# Autodesk Inventor assembly: Milestione One Assembly
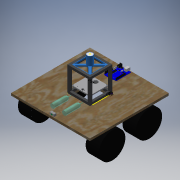
[picture p0: Inventor's stored thumbnail of the model, 180x180]
Saved by Autodesk Inventor 2016 (Build 200138000, 138)
## iProperties
Created: 2016-02-22
Part Number: Milestione One Assembly
Document SubType Name: Assembly
Designer: Kenneth Daniel
Author: Kenneth Daniel
## Documents named in this file (12)
- C:\Users\Kenneth Daniel\Documents\Enes 100A\CAD Assignments\Milestione One Assembly.iam
- C:\Users\Kenneth Daniel\Documents\Enes 100A\Bassic Vehicle Chassis.ipt
- C:\Users\Kenneth Daniel\Documents\Enes 100A\Lifting Main Frame.ipt
- C:\Users\Kenneth Daniel\Documents\Enes 100A\Motor housing for Lifting Platform.ipt
- C:\Users\Kenneth Daniel\Documents\Enes 100A\Moving Surface.ipt
- C:\Users\Kenneth Daniel\Documents\Enes 100A\Syringe Ken.ipt
- C:\Users\Kenneth Daniel\Documents\Enes 100A\CAD Assignments\Lifting Pad Motor Redo.ipt
- C:\Users\Kenneth Daniel\Documents\Enes 100A\CAD Assignments\Wheel Holder.ipt
- C:\Users\Kenneth Daniel\Documents\Enes 100A\CAD Assignments\Susspension Holder.ipt
- C:\Users\Kenneth Daniel\Documents\Enes 100A\CAD Assignments\Basic OSV Wheel.ipt
- C:\Users\Kenneth Daniel\Documents\Enes 100A\arduino uno.iam
- C:\Users\Kenneth Daniel\Documents\Enes 100A\CAD Assignments\Basic Sensor.ipt
## Components (25 placed, 11 different names)
1. Bassic Vehicle Chassis:1 — Mate:3, Mate:4, Mate:5, Mate:10, Mate:11, Mate:12, Mate:13, Mate:14, Mate:15, Mate:16, Mate:17, Mate:18, Mate:19, Mate:20, Mate:21, Mate:22, Mate:23, Mate:24, Mate:25, Mate:26, Mate:47
2. Lifting Main Frame:1 — Mate:1, Mate:2, Mate:3, Mate:4, Mate:5, Mate:6, Mate:7, Mate:8
3. Motor housing for Lifting Platform:1 — Mate:1, Mate:2, Mate:6, Mate:9
4. Moving Surface:1 — Mate:7, Mate:8
5. Syringe Ken:1
6. Syringe Ken:2
7. Lifting Pad Motor Redo:1 — Mate:9
8. Wheel Holder:1 — Mate:13, Mate:29, Mate:32, Mate:34, Mate:41, Mate:42
9. Wheel Holder:2 — Mate:12, Mate:28, Mate:37, Mate:38, Mate:45, Mate:46
10. Wheel Holder:3 — Mate:11, Mate:26, Mate:27, Mate:35, Mate:36, Mate:43, Mate:44
11. Wheel Holder:4 — Mate:10, Mate:30, Mate:31, Mate:33, Mate:39, Mate:40
12. Susspension Holder:1 — Mate:14, Mate:15, Mate:16, Mate:30
13. Susspension Holder:2 — Mate:17, Mate:18, Mate:19, Mate:29
14. Susspension Holder:3 — Mate:20, Mate:21, Mate:22, Mate:27
15. Susspension Holder:4 — Mate:23, Mate:24, Mate:25, Mate:28
16. Basic OSV Wheel:1 — Mate:31, Mate:33
17. Basic OSV Wheel:2 — Mate:35, Mate:36
18. Basic OSV Wheel:3 — Mate:32, Mate:34
19. Basic OSV Wheel:4 — Mate:37, Mate:38
20. Lifting Pad Motor Redo:2 — Mate:41, Mate:42
21. Lifting Pad Motor Redo:3 — Mate:39, Mate:40
22. Lifting Pad Motor Redo:4 — Mate:43, Mate:44
23. Lifting Pad Motor Redo:5 — Mate:45, Mate:46
24. arduino uno:1 [sub-assembly]
25. Basic Sensor:1 — Mate:47
## Relationships (47: Mate 47)
- Mate:1: Lifting Main Frame:1 ↔ Motor housing for Lifting Platform:1
- Mate:2: Lifting Main Frame:1 ↔ Motor housing for Lifting Platform:1
- Mate:3: Bassic Vehicle Chassis:1 ↔ Lifting Main Frame:1
- Mate:4: Bassic Vehicle Chassis:1 ↔ Lifting Main Frame:1
- Mate:5: Bassic Vehicle Chassis:1 ↔ Lifting Main Frame:1
- Mate:6: Lifting Main Frame:1 ↔ Motor housing for Lifting Platform:1
- Mate:7: Lifting Main Frame:1 ↔ Moving Surface:1
- Mate:8: Lifting Main Frame:1 ↔ Moving Surface:1
- Mate:9: Motor housing for Lifting Platform:1 ↔ Lifting Pad Motor Redo:1
- Mate:10: Bassic Vehicle Chassis:1 ↔ Wheel Holder:4
- Mate:11: Bassic Vehicle Chassis:1 ↔ Wheel Holder:3
- Mate:12: Bassic Vehicle Chassis:1 ↔ Wheel Holder:2
- Mate:13: Bassic Vehicle Chassis:1 ↔ Wheel Holder:1
- Mate:14: Bassic Vehicle Chassis:1 ↔ Susspension Holder:1
- Mate:15: Bassic Vehicle Chassis:1 ↔ Susspension Holder:1
- Mate:16: Bassic Vehicle Chassis:1 ↔ Susspension Holder:1
- Mate:17: Bassic Vehicle Chassis:1 ↔ Susspension Holder:2
- Mate:18: Bassic Vehicle Chassis:1 ↔ Susspension Holder:2
- Mate:19: Bassic Vehicle Chassis:1 ↔ Susspension Holder:2
- Mate:20: Bassic Vehicle Chassis:1 ↔ Susspension Holder:3
- Mate:21: Bassic Vehicle Chassis:1 ↔ Susspension Holder:3
- Mate:22: Bassic Vehicle Chassis:1 ↔ Susspension Holder:3
- Mate:23: Bassic Vehicle Chassis:1 ↔ Susspension Holder:4
- Mate:24: Bassic Vehicle Chassis:1 ↔ Susspension Holder:4
- Mate:25: Bassic Vehicle Chassis:1 ↔ Susspension Holder:4
- Mate:26: Bassic Vehicle Chassis:1 ↔ Wheel Holder:3
- Mate:27: Wheel Holder:3 ↔ Susspension Holder:3
- Mate:28: Wheel Holder:2 ↔ Susspension Holder:4
- Mate:29: Wheel Holder:1 ↔ Susspension Holder:2
- Mate:30: Wheel Holder:4 ↔ Susspension Holder:1
- Mate:31: Wheel Holder:4 ↔ Basic OSV Wheel:1
- Mate:32: Wheel Holder:1 ↔ Basic OSV Wheel:3
- Mate:33: Wheel Holder:4 ↔ Basic OSV Wheel:1
- Mate:34: Wheel Holder:1 ↔ Basic OSV Wheel:3
- Mate:35: Wheel Holder:3 ↔ Basic OSV Wheel:2
- Mate:36: Wheel Holder:3 ↔ Basic OSV Wheel:2
- Mate:37: Wheel Holder:2 ↔ Basic OSV Wheel:4
- Mate:38: Wheel Holder:2 ↔ Basic OSV Wheel:4
- Mate:39: Wheel Holder:4 ↔ Lifting Pad Motor Redo:3
- Mate:40: Wheel Holder:4 ↔ Lifting Pad Motor Redo:3
- Mate:41: Wheel Holder:1 ↔ Lifting Pad Motor Redo:2
- Mate:42: Wheel Holder:1 ↔ Lifting Pad Motor Redo:2
- Mate:43: Wheel Holder:3 ↔ Lifting Pad Motor Redo:4
- Mate:44: Wheel Holder:3 ↔ Lifting Pad Motor Redo:4
- Mate:45: Wheel Holder:2 ↔ Lifting Pad Motor Redo:5
- Mate:46: Wheel Holder:2 ↔ Lifting Pad Motor Redo:5
- Mate:47: Bassic Vehicle Chassis:1 ↔ Basic Sensor:1
